# Autodesk Inventor assembly: mb_mother_board
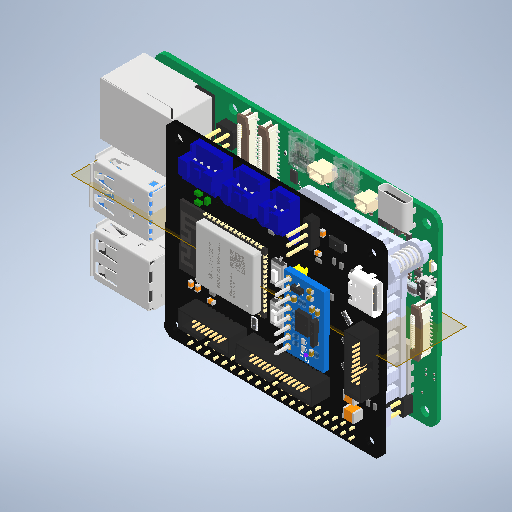
[picture p0: Inventor's stored thumbnail of the model, 512x512]
Saved by Autodesk Inventor 2025 (Build 290162000, 162)
## iProperties
Created: 2026-07-21
Part Number: mb_mother_board
Document SubType Name: Assembly
Designer: garin
Author: garin
## Documents named in this file (18)
- C:\Users\Leva\Documents\Git\TheseusV2_Maze\Construction\Theseus_v2\mother_board\mb_mother_board.iam
- C:\Users\Leva\Documents\Git\TheseusV2_Maze\Construction\Theseus_v2\mother_board\CONB127P-2R-14W_TH.ipt
- C:\Users\Leva\Documents\Git\TheseusV2_Maze\Construction\Theseus_v2\mother_board\ESP32-S3-WROOM.ipt
- C:\Users\Leva\Documents\Git\TheseusV2_Maze\Construction\Theseus_v2\mother_board\rpi-5b_no_graphics.ipt
- C:\Users\Leva\Documents\Git\TheseusV2_Maze\Construction\Theseus_v2\mother_board\PBD-40.ipt
- C:\Users\garin\Documents\models\altium_models\pls_connectors\PLS-3\PLS-3.ipt
- C:\Users\Leva\Documents\Git\TheseusV2_Maze\Construction\Theseus_v2\mother_board\Heatsink+fan RPi-5.ipt
- C:\Users\Leva\Documents\Git\TheseusV2_Maze\Construction\Theseus_v2\mother_board\S03B-PASK-2.ipt
- C:\Users\Leva\Documents\Git\TheseusV2_Maze\Construction\Theseus_v2\mother_board\S04B-PASK-2.ipt
- C:\Users\garin\Documents\Git\TheseusV2_Maze\Construction\Theseus_v2\B02B-PASK\B02B-PASK.ipt
- C:\Users\Leva\Documents\Git\TheseusV2_Maze\Construction\Theseus_v2\mother_board\CONB127P-2R-10W_TH.ipt
- C:\Users\Leva\Documents\Git\TheseusV2_Maze\Construction\Theseus_v2\mother_board\board_rpi.ipt
- C:\Users\Leva\Documents\Git\TheseusV2_Maze\Construction\Theseus_v2\mother_board\CMUCF661030E.ipt
- C:\Users\Leva\Documents\Git\TheseusV2_Maze\Construction\Theseus_v2\mother_board\GY-BNO055.ipt
- C:\Users\garin\Documents\models\altium_models\pls_connectors\PLS-8\PLS-8.ipt
- C:\Users\Leva\Documents\Git\TheseusV2_Maze\Construction\Theseus_v2\S02B-PASK-2.ipt
- C:\Users\Leva\Documents\Git\TheseusV2_Maze\Construction\Theseus_v2\mother_board\CONB127P-2R-26W_TH.ipt
- C:\Users\Leva\Documents\Git\TheseusV2_Maze\Schematic\TSE_mother_board\TSE_mother_board_1.ipt
## Components (20 placed, 17 different names)
1. CONB127P-2R-14W_TH:1 — Совмещение:12, Заподлицо:12, Совмещение:44, Совмещение:45
2. rpi-5b_no_graphics:1 — Совмещение:1, Совмещение:2, Угол:1, Совмещение:4, Заподлицо:3, Заподлицо:4, Совмещение:52, Совмещение:53, Совмещение:54
3. PBD-40:1 — Заподлицо:1, Совмещение:3, Заподлицо:2, Совмещение:4, Заподлицо:3, Заподлицо:4, Совмещение:8, Совмещение:31, Совмещение:36, Совмещение:50
4. Heatsink+fan RPi-5:1 — Совмещение:1, Совмещение:2, Угол:1
5. S03B-PASK-2:1 — Совмещение:25, Заподлицо:21, Совмещение:26, Совмещение:29, Совмещение:48
6. S04B-PASK-2:1 — Совмещение:23, Заподлицо:20, Заподлицо:34, Совмещение:26
7. CONB127P-2R-10W_TH:1 — Совмещение:7, Совмещение:8, Заподлицо:33, Совмещение:51
8. board_rpi:1 — Заподлицо:1, Совмещение:3, Заподлицо:2, Совмещение:7, Совмещение:12, Заподлицо:12, Совмещение:18, Заподлицо:16, Совмещение:20, Заподлицо:17, Совмещение:23, Заподлицо:20, Совмещение:25, Заподлицо:21, Совмещение:27, Заподлицо:22, Заподлицо:23, Совмещение:28, Заподлицо:24, Совмещение:30, Заподлицо:25, Совмещение:35, Совмещение:38, Заподлицо:26, Совмещение:40, Совмещение:44, Заподлицо:33, Заподлицо:34, Совмещение:47, Заподлицо:35, Совмещение:49
9. B02B-PASK:3 — Совмещение:18, Заподлицо:16, Совмещение:33
10. ESP32-S3-WROOM:1 — Совмещение:20, Заподлицо:17, Совмещение:41, Совмещение:46
11. PLS-3:1 — Совмещение:28, Заподлицо:24, Совмещение:29, Совмещение:33
12. B02B-PASK:5 — Совмещение:30, Совмещение:31, Заподлицо:25, Совмещение:46
13. B02B-PASK:6 — Совмещение:27, Заподлицо:22, Заподлицо:23
14. B02B-PASK:7 — Совмещение:35, Совмещение:36
15. CMUCF661030E:1 — Совмещение:38, Заподлицо:26, Совмещение:45
16. GY-BNO055:1 — Совмещение:43, Заподлицо:27, Заподлицо:28
17. PLS-8:1 — Совмещение:40, Совмещение:41, Совмещение:43, Заподлицо:27, Заподлицо:28
18. S02B-PASK-2:1 — Совмещение:47, Заподлицо:35, Совмещение:48
19. CONB127P-2R-26W_TH:1 — Совмещение:49, Совмещение:50, Совмещение:51
20. TSE_mother_board_1:1 — Совмещение:52, Совмещение:53, Совмещение:54
## Relationships (55: Mate 35, Flush 19, Angle 1)
- Совмещение:1 [Mate]: rpi-5b_no_graphics:1 ↔ Heatsink+fan RPi-5:1
- Совмещение:2 [Mate]: rpi-5b_no_graphics:1 ↔ Heatsink+fan RPi-5:1
- Угол:1 [Angle] (0 deg): rpi-5b_no_graphics:1 ↔ Heatsink+fan RPi-5:1
- Заподлицо:1 [Flush] (-0.96 mm): PBD-40:1 ↔ board_rpi:1
- Совмещение:3 [Mate]: PBD-40:1 ↔ board_rpi:1
- Заподлицо:2 [Flush] (-7.1 mm): PBD-40:1 ↔ board_rpi:1
- Совмещение:4 [Mate] (3 mm): rpi-5b_no_graphics:1 ↔ PBD-40:1
- Заподлицо:3 [Flush]: rpi-5b_no_graphics:1 ↔ PBD-40:1
- Заподлицо:4 [Flush]: rpi-5b_no_graphics:1 ↔ PBD-40:1
- Совмещение:7 [Mate]: CONB127P-2R-10W_TH:1 ↔ board_rpi:1
- Совмещение:8 [Mate] (3 mm): PBD-40:1 ↔ CONB127P-2R-10W_TH:1
- Совмещение:12 [Mate]: CONB127P-2R-14W_TH:1 ↔ board_rpi:1
- Заподлицо:12 [Flush] (-17.405 mm): CONB127P-2R-14W_TH:1 ↔ board_rpi:1
- Совмещение:18 [Mate]: board_rpi:1 ↔ B02B-PASK:3
- Заподлицо:16 [Flush]: board_rpi:1 ↔ B02B-PASK:3
- Совмещение:20 [Mate]: board_rpi:1 ↔ ESP32-S3-WROOM:1
- Заподлицо:17 [Flush] (5 mm): board_rpi:1 ↔ ESP32-S3-WROOM:1
- Совмещение:23 [Mate]: S04B-PASK-2:1 ↔ board_rpi:1
- Заподлицо:20 [Flush]: S04B-PASK-2:1 ↔ board_rpi:1
- Заподлицо:34 [Flush] (10 mm): S04B-PASK-2:1 ↔ board_rpi:1
- Совмещение:25 [Mate]: S03B-PASK-2:1 ↔ board_rpi:1
- Заподлицо:21 [Flush]: S03B-PASK-2:1 ↔ board_rpi:1
- Совмещение:26 [Mate] (3 mm): S03B-PASK-2:1 ↔ S04B-PASK-2:1
- Совмещение:27 [Mate]: board_rpi:1 ↔ B02B-PASK:6
- Заподлицо:22 [Flush]: board_rpi:1 ↔ B02B-PASK:6
- Заподлицо:23 [Flush] (7.705 mm): board_rpi:1 ↔ B02B-PASK:6
- Совмещение:28 [Mate]: board_rpi:1 ↔ PLS-3:1
- Заподлицо:24 [Flush] (3 mm): board_rpi:1 ↔ PLS-3:1
- Совмещение:29 [Mate] (3 mm): S03B-PASK-2:1 ↔ PLS-3:1
- Совмещение:30 [Mate]: board_rpi:1 ↔ B02B-PASK:5
- Совмещение:31 [Mate] (3 mm): PBD-40:1 ↔ B02B-PASK:5
- Заподлицо:25 [Flush] (5 mm): board_rpi:1 ↔ B02B-PASK:5
- Заподлицо:33 [Flush] (10 mm): CONB127P-2R-10W_TH:1 ↔ board_rpi:1
- Совмещение:33 [Mate] (3 mm): B02B-PASK:3 ↔ PLS-3:1
- Совмещение:35 [Mate]: board_rpi:1 ↔ B02B-PASK:7
- Совмещение:36 [Mate] (3 mm): PBD-40:1 ↔ B02B-PASK:7
- Совмещение:38 [Mate]: board_rpi:1 ↔ CMUCF661030E:1
- Заподлицо:26 [Flush] (1 mm): board_rpi:1 ↔ CMUCF661030E:1
- Совмещение:40 [Mate]: board_rpi:1 ↔ PLS-8:1
- Совмещение:41 [Mate] (10 mm): ESP32-S3-WROOM:1 ↔ PLS-8:1
- Совмещение:43 [Mate]: GY-BNO055:1 ↔ PLS-8:1
- Заподлицо:27 [Flush]: GY-BNO055:1 ↔ PLS-8:1
- Заподлицо:28 [Flush]: GY-BNO055:1 ↔ PLS-8:1
- Совмещение:44 [Mate] (2 mm): CONB127P-2R-14W_TH:1 ↔ board_rpi:1
- Совмещение:45 [Mate] (3 mm): CONB127P-2R-14W_TH:1 ↔ CMUCF661030E:1
- Совмещение:46 [Mate] (6.615 mm): ESP32-S3-WROOM:1 ↔ B02B-PASK:5
- Совмещение:47 [Mate]: board_rpi:1 ↔ S02B-PASK-2:1
- Заподлицо:35 [Flush]: board_rpi:1 ↔ S02B-PASK-2:1
- Совмещение:48 [Mate] (3 mm): S03B-PASK-2:1 ↔ S02B-PASK-2:1
- Совмещение:49 [Mate]: board_rpi:1 ↔ CONB127P-2R-26W_TH:1
- Совмещение:50 [Mate] (3 mm): PBD-40:1 ↔ CONB127P-2R-26W_TH:1
- Совмещение:51 [Mate] (2 mm): CONB127P-2R-10W_TH:1 ↔ CONB127P-2R-26W_TH:1
- Совмещение:52 [Mate]: rpi-5b_no_graphics:1 ↔ TSE_mother_board_1:1
- Совмещение:53 [Mate]: rpi-5b_no_graphics:1 ↔ TSE_mother_board_1:1
- Совмещение:54 [Mate] (15 mm): rpi-5b_no_graphics:1 ↔ TSE_mother_board_1:1
